# Autodesk Inventor assembly: 145
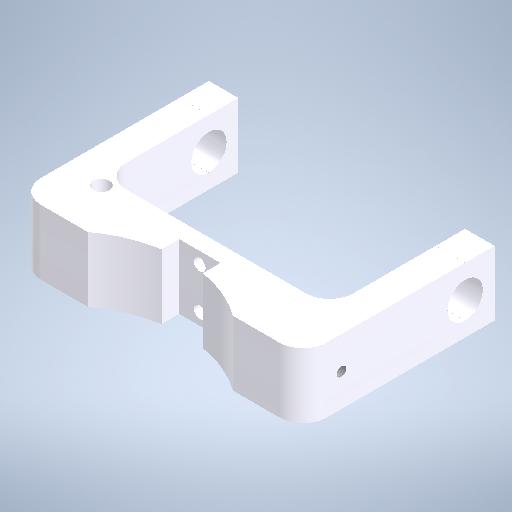
[picture p0: Inventor's stored thumbnail of the model, 512x512]
Saved by Autodesk Inventor 2025.1 (Build 291241000, 241)
## iProperties
Created: 2024-08-01
Part Number: 145
Document SubType Name: Assembly
Designer: ffogue
Author: ffogue
## Documents named in this file (4)
- C:\Projkete - Übungen\Freedom\145.iam
- C:\Projkete - Übungen\Freedom\145 part 2.ipt
- C:\Projkete - Übungen\Freedom\145 part.ipt
- C:\Projkete - Übungen\Freedom\145 part_MIR2.ipt
## Components (3 placed, 3 different names)
1. 145 part 2:1 — Fluchtend:1
2. 145 part:1 — Fluchtend:1
3. 145 part_MIR2:1
## Relationships (2: Flush 2)
- Fluchtend:1 [Flush]: 145 part 2:1 ↔ 145 part:1
- Fluchtend:2 [Flush] (-6 mm)
